# Autodesk Inventor assembly: Helenowiak
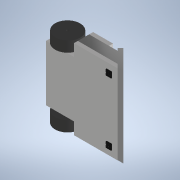
[picture p0: Inventor's stored thumbnail of the model, 180x180]
Saved by Autodesk Inventor 2021 (Build 250183000, 183)
## iProperties
Created: 2021-03-30
Part Number: Helenowiak
Document SubType Name: Assembly
Designer: jakub
Author: jakub
## Documents named in this file (13)
- E:\Projekty\Minisumo Helenowiak\Helenowiak\Helenowiak_mechanika\Helenowiak.iam
- E:\Projekty\Minisumo Helenowiak\Helenowiak\Helenowiak_mechanika\Helenowiak_podstawa.ipt
- E:\Projekty\Minisumo Helenowiak\Helenowiak\Helenowiak_mechanika\Helenowiak_plug.ipt
- E:\Projekty\Minisumo Helenowiak\Helenowiak\Helenowiak_mechanika\micro-metal-gearmotor-extended-with-1086-bracket.ipt
- E:\Projekty\Minisumo Helenowiak\Helenowiak\Helenowiak_mechanika\Kolo_Pololu1127.ipt
- E:\Projekty\Minisumo Helenowiak\Helenowiak\Helenowiak_mechanika\magnetic-encoder-pair-kit-for-micro-metal-gearmotors-hpcb-compatible-enc03b.ipt
- E:\Projekty\Minisumo Helenowiak\Helenowiak\Helenowiak_mechanika\magnetic-encoder-pair-kit-for-micro-metal-gearmotors-hpcb-compatible-w1r02a.ipt
- E:\Projekty\Minisumo Helenowiak\Helenowiak\Helenowiak_mechanika\cny70.ipt
- E:\Projekty\Minisumo Helenowiak\Helenowiak\Helenowiak_mechanika\Polulu2578pololu-38-khz-ir-proximity-sensor.ipt
- E:\Projekty\Minisumo Helenowiak\Helenowiak\Helenowiak_mechanika\LiPol.ipt
- E:\Projekty\Minisumo Helenowiak\Helenowiak\Helenowiak_mechanika\Helenowiak_sciana.ipt
- E:\Projekty\Minisumo Helenowiak\Helenowiak\Helenowiak_mechanika\Helenowiak_polka.ipt
- E:\Projekty\Minisumo Helenowiak\Helenowiak\Helenowiak_mechanika\PCB.ipt
## Components (19 placed, 12 different names)
1. Helenowiak_podstawa:1 — Zestawiające:5, Zestawiające:9, Zestawiające:10, Równoległe:6, Równoległe:7, Równoległe:8, Równoległe:9, Równoległe:10, Równoległe:11, Zestawiające:14, Zestawiające:15, Zestawiające:20, Równoległe:12, Zestawiające:21, Równoległe:13, Równoległe:17
2. Helenowiak_plug:1 — Zestawiające:5, Równoległe:9, Zestawiające:19, Zestawiające:22, Równoległe:17
3. micro-metal-gearmotor-extended-with-1086-bracket:1 — Zestawiające:8, Zestawiające:10, Równoległe:7, Zestawiające:11, Wstawiające:2, Wstawiające:4
4. micro-metal-gearmotor-extended-with-1086-bracket:2 — Zestawiające:6, Zestawiające:7, Zestawiające:9, Równoległe:6, Zestawiające:11, Wstawiające:1, Wstawiające:3
5. Kolo_Pololu1127:1 — Zestawiające:6, Zestawiające:7, Równoległe:8
6. Kolo_Pololu1127:2 — Zestawiające:8
7. magnetic-encoder-pair-kit-for-micro-metal-gearmotors-hpcb-compatible-enc03b:1 — Wstawiające:1
8. magnetic-encoder-pair-kit-for-micro-metal-gearmotors-hpcb-compatible-enc03b:2 — Wstawiające:2
9. magnetic-encoder-pair-kit-for-micro-metal-gearmotors-hpcb-compatible-w1r02a:1 — Wstawiające:4
10. magnetic-encoder-pair-kit-for-micro-metal-gearmotors-hpcb-compatible-w1r02a:2 — Wstawiające:3
11. cny70:4 — Równoległe:10
12. cny70:5 — Równoległe:11
13. Polulu2578pololu-38-khz-ir-proximity-sensor:1 — Zestawiające:15
14. Polulu2578pololu-38-khz-ir-proximity-sensor:2 — Zestawiające:14
15. LiPol:1 — Zestawiające:25, Równoległe:18
16. Podpora:4 — Zestawiające:19, Zestawiające:20, Równoległe:12, Zestawiające:24, Równoległe:16
17. Podpora:5 — Zestawiające:21, Zestawiające:22, Równoległe:13, Równoległe:15
18. Helenowiak_Polka:1 — Zestawiające:24, Równoległe:15, Równoległe:16, Zestawiające:25, Równoległe:18
19. PCB:1
## Relationships (31: Mate 15, Flush 12, Insert 4)
- Zestawiające:5 [Mate]: Helenowiak_podstawa:1 ↔ Helenowiak_plug:1
- Zestawiające:6 [Mate]: micro-metal-gearmotor-extended-with-1086-bracket:2 ↔ Kolo_Pololu1127:1
- Zestawiające:7 [Mate]: micro-metal-gearmotor-extended-with-1086-bracket:2 ↔ Kolo_Pololu1127:1
- Zestawiające:8 [Mate]: micro-metal-gearmotor-extended-with-1086-bracket:1 ↔ Kolo_Pololu1127:2
- Zestawiające:9 [Mate]: Helenowiak_podstawa:1 ↔ micro-metal-gearmotor-extended-with-1086-bracket:2
- Zestawiające:10 [Mate]: Helenowiak_podstawa:1 ↔ micro-metal-gearmotor-extended-with-1086-bracket:1
- Równoległe:6 [Flush]: Helenowiak_podstawa:1 ↔ micro-metal-gearmotor-extended-with-1086-bracket:2
- Równoległe:7 [Flush]: Helenowiak_podstawa:1 ↔ micro-metal-gearmotor-extended-with-1086-bracket:1
- Równoległe:8 [Flush]: Helenowiak_podstawa:1 ↔ Kolo_Pololu1127:1
- Zestawiające:11 [Mate]: micro-metal-gearmotor-extended-with-1086-bracket:1 ↔ micro-metal-gearmotor-extended-with-1086-bracket:2
- Równoległe:9 [Flush]: Helenowiak_podstawa:1 ↔ Helenowiak_plug:1
- Wstawiające:1 [Insert]: micro-metal-gearmotor-extended-with-1086-bracket:2 ↔ magnetic-encoder-pair-kit-for-micro-metal-gearmotors-hpcb-compatible-enc03b:1
- Wstawiające:2 [Insert]: micro-metal-gearmotor-extended-with-1086-bracket:1 ↔ magnetic-encoder-pair-kit-for-micro-metal-gearmotors-hpcb-compatible-enc03b:2
- Wstawiające:3 [Insert]: micro-metal-gearmotor-extended-with-1086-bracket:2 ↔ magnetic-encoder-pair-kit-for-micro-metal-gearmotors-hpcb-compatible-w1r02a:2
- Wstawiające:4 [Insert]: micro-metal-gearmotor-extended-with-1086-bracket:1 ↔ magnetic-encoder-pair-kit-for-micro-metal-gearmotors-hpcb-compatible-w1r02a:1
- Równoległe:10 [Flush]: Helenowiak_podstawa:1 ↔ cny70:4
- Równoległe:11 [Flush]: Helenowiak_podstawa:1 ↔ cny70:5
- Zestawiające:14 [Mate]: Helenowiak_podstawa:1 ↔ Polulu2578pololu-38-khz-ir-proximity-sensor:2
- Zestawiające:15 [Mate]: Helenowiak_podstawa:1 ↔ Polulu2578pololu-38-khz-ir-proximity-sensor:1
- Zestawiające:19 [Mate]: Helenowiak_plug:1 ↔ Podpora:4
- Zestawiające:20 [Mate]: Helenowiak_podstawa:1 ↔ Podpora:4
- Równoległe:12 [Flush]: Helenowiak_podstawa:1 ↔ Podpora:4
- Zestawiające:21 [Mate]: Helenowiak_podstawa:1 ↔ Podpora:5
- Zestawiające:22 [Mate]: Helenowiak_plug:1 ↔ Podpora:5
- Równoległe:13 [Flush]: Helenowiak_podstawa:1 ↔ Podpora:5
- Zestawiające:24 [Mate]: Podpora:4 ↔ Helenowiak_Polka:1
- Równoległe:15 [Flush]: Podpora:5 ↔ Helenowiak_Polka:1
- Równoległe:16 [Flush]: Podpora:4 ↔ Helenowiak_Polka:1
- Równoległe:17 [Flush]: Helenowiak_podstawa:1 ↔ Helenowiak_plug:1
- Zestawiające:25 [Mate]: LiPol:1 ↔ Helenowiak_Polka:1
- Równoległe:18 [Flush]: LiPol:1 ↔ Helenowiak_Polka:1
